# Autodesk Inventor assembly: Assembly1
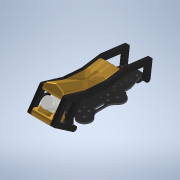
[picture p0: Inventor's stored thumbnail of the model, 180x180]
Saved by Autodesk Inventor 2020 (Build 240168000, 168)
## iProperties
Created: 2022-05-03
Part Number: Assembly1
Document SubType Name: Assembly
Designer: Steven
Author: Steven
## Documents named in this file (8)
- Y:\FPV drone stuff\0 Street League\Frames\PB-Kauri-X\3D prints\35 mm canopy\Assembly1.iam
- Y:\FPV drone stuff\0 Street League\Frames\PB-Kauri-X\Kauri side plate.ipt
- Y:\FPV drone stuff\0 Street League\Frames\PB-Kauri-X\3D prints\35 mm canopy\KauriCanopy Pb.ipt
- Y:\FPV drone stuff\0 Street League\Frames\PB-Kauri-X\Kauri mid plate v2.ipt
- Y:\FPV drone stuff\0 Street League\Frames\PB-Kauri-X\3D prints\35 mm canopy\KauriFrontLink 35mm.ipt
- Y:\FPV drone stuff\0 Street League\Frames\PB-Kauri-X\3D prints\35 mm canopy\KauriRearLink 35mm no brass insert.ipt
- Y:\FPV drone stuff\0 Street League\Frames\PB-Kauri-X\3D prints\35 mm canopy\35mm standoff.ipt
- Y:\FPV drone stuff\0 Street League\Frames\PB-Kauri-X\3D prints\35 mm canopy\predator mini cam standoff mount.iam
## Components (9 placed, 7 different names)
1. Kauri side plate:1 — Insert:2, Insert:4, Insert:5, Insert:6
2. Kauri side plate:2 — Insert:1, Insert:3, Insert:9, Insert:10, Mate:2, Insert:11, Insert:12, Mate:3
3. KauriCanopy Pb:1 — Insert:1, Insert:2, Insert:3, Insert:4
4. KauriFrontLink 35mm:1 — Insert:5, Flush:1, Mate:1, Insert:7
5. KauriRearLink 35mm no brass insert:1 — Insert:6, Flush:1, Insert:8
6. Kauri mid plate v2:1 — Mate:1, Insert:7, Insert:8
7. 35mm standoff:1 — Insert:9
8. 35mm standoff:2 — Insert:10
9. predator mini cam standoff mount:1 [sub-assembly] — Mate:2, Insert:11, Insert:12
## Relationships (16: Insert 12, Mate 3, Flush 1)
- Insert:1: Kauri side plate:2 ↔ KauriCanopy Pb:1
- Insert:2: Kauri side plate:1 ↔ KauriCanopy Pb:1
- Insert:3: Kauri side plate:2 ↔ KauriCanopy Pb:1
- Insert:4: Kauri side plate:1 ↔ KauriCanopy Pb:1
- Insert:5: Kauri side plate:1 ↔ KauriFrontLink 35mm:1
- Insert:6: Kauri side plate:1 ↔ KauriRearLink 35mm no brass insert:1
- Flush:1: KauriFrontLink 35mm:1 ↔ KauriRearLink 35mm no brass insert:1
- Mate:1: KauriFrontLink 35mm:1 ↔ Kauri mid plate v2:1
- Insert:7: KauriFrontLink 35mm:1 ↔ Kauri mid plate v2:1
- Insert:8: KauriRearLink 35mm no brass insert:1 ↔ Kauri mid plate v2:1
- Insert:9: Kauri side plate:2 ↔ 35mm standoff:1
- Insert:10: Kauri side plate:2 ↔ 35mm standoff:2
- Mate:2: Kauri side plate:2 ↔ predator mini cam standoff mount:1
- Insert:11: Kauri side plate:2 ↔ predator mini cam standoff mount:1
- Insert:12: Kauri side plate:2 ↔ predator mini cam standoff mount:1
- Mate:3: Kauri side plate:2
